# Autodesk Inventor assembly: ЛЦМК000002.00.00.00.02.00 Правое крепление
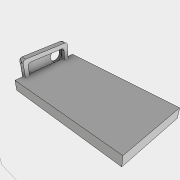
[picture p0: Inventor's stored thumbnail of the model, 180x180]
Saved by Autodesk Inventor 2021.2 (Build 252289000, 289)
## iProperties
Created: 2025-11-09
Part Number: ЛЦМК000002.00.00.00.02.00 Правое крепление
Document SubType Name: Assembly
Designer: Захаров
Author: Захаров
## Documents named in this file (3)
- C:\Users\User\Documents\CaseARHead1\ЛЦМК000002.00.00.00.02.00 Правое крепление.iam
- C:\Users\User\Documents\CaseARHead1\ЛЦМК000002.00.00.00.00.15.ipt
- C:\Users\User\Documents\CaseARHead1\ЛЦМК000002.00.00.00.00.17.ipt
## Components (2 placed, 2 different names)
1. ЛЦМК000002.00.00.00.00.15:1 — Заподлицо:1, Заподлицо:2, Совмещение:1
2. ЛЦМК000002.00.00.00.00.17:1 — Заподлицо:1, Заподлицо:2, Совмещение:1
## Relationships (3: Flush 2, Mate 1)
- Заподлицо:1 [Flush]: ЛЦМК000002.00.00.00.00.15:1 ↔ ЛЦМК000002.00.00.00.00.17:1
- Заподлицо:2 [Flush]: ЛЦМК000002.00.00.00.00.15:1 ↔ ЛЦМК000002.00.00.00.00.17:1
- Совмещение:1 [Mate] (-2 mm): ЛЦМК000002.00.00.00.00.15:1 ↔ ЛЦМК000002.00.00.00.00.17:1
